# Autodesk Inventor assembly: ClockFace
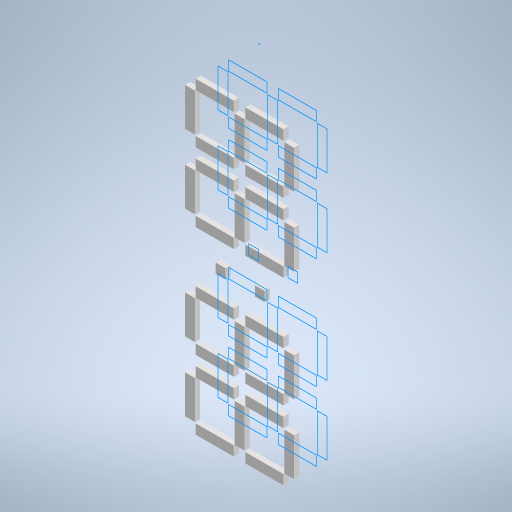
[picture p0: Inventor's stored thumbnail of the model, 512x512]
Saved by Autodesk Inventor 2024.2 (Build 282272000, 272)
## iProperties
Created: 2024-01-22
Part Number: ClockFace
Document SubType Name: Assembly
Designer: Felix
Author: Felix
## Documents named in this file (4)
- D:\Programmieren\LedClock\Inventor\ClockFace.iam
- D:\Programmieren\LedClock\Inventor\Digit.ipt
- D:\Programmieren\LedClock\Inventor\Dots2.ipt
- D:\Programmieren\LedClock\Inventor\drawing.ipt
## Components (6 placed, 3 different names)
1. Digit:2 — Flush:3, Flush:6, Mate:1
2. Digit:3 — Flush:2, Flush:5, Mate:1, Mate:2
3. Digit:4 — Flush:1, Flush:4, Flush:7, Mate:3, Mate:4
4. Digit:5 — Flush:1, Flush:2, Flush:3, Flush:4, Flush:5, Flush:6, Mate:4
5. Dots2:1 — Flush:7, Mate:2, Mate:3
6. drawing:1
## Relationships (11: Flush 7, Mate 4)
- Flush:1: Digit:4 ↔ Digit:5
- Flush:2: Digit:3 ↔ Digit:5
- Flush:3: Digit:2 ↔ Digit:5
- Flush:4: Digit:4 ↔ Digit:5
- Flush:5: Digit:3 ↔ Digit:5
- Flush:6: Digit:2 ↔ Digit:5
- Flush:7: Digit:4 ↔ Dots2:1
- Mate:1 (17 mm): Digit:2 ↔ Digit:3
- Mate:2 (36 mm): Digit:3 ↔ Dots2:1
- Mate:3 (36 mm): Digit:4 ↔ Dots2:1
- Mate:4 (17 mm): Digit:4 ↔ Digit:5
## Named parameters: KERNING = 17 mm, DOTKERN = -19 mm
